# Autodesk Inventor assembly: fork_left
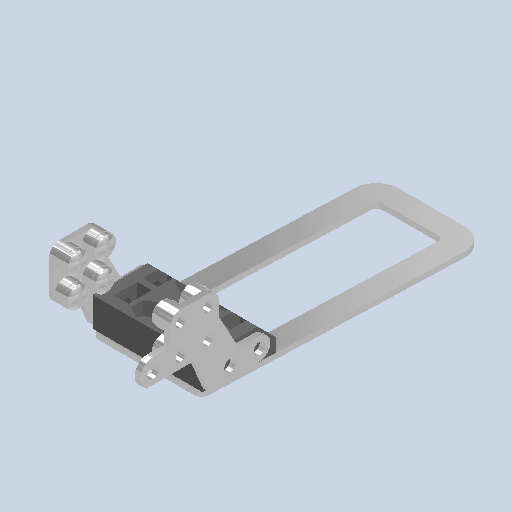
[picture p0: Inventor's stored thumbnail of the model, 512x512]
Saved by Autodesk Inventor 2024.1 (Build 281209000, 209)
## iProperties
Created: 2025-01-18
Part Number: fork_left
Document SubType Name: Assembly
Designer: hibik
Author: hibik
## Documents named in this file (6)
- C:\Users\hibik\Documents\Robomech\RESCUE\ORCA\hard\fork\left\fork_left.iam
- C:\Users\hibik\Documents\Robomech\RESCUE\ORCA\hard\fork\left\fork_middle_left.ipt
- C:\Users\hibik\Documents\Robomech\RESCUE\ORCA\hard\fork\left\fork_inside_left.ipt
- C:\Users\hibik\Documents\Robomech\RESCUE\ORCA\hard\fork\left\fork_outside_left.ipt
- C:\Users\hibik\Documents\Robomech\RESCUE\ORCA\hard\fork\left\bearing_3_6_2.5_left.ipt
- C:\Users\hibik\Documents\Robomech\RESCUE\ORCA\hard\fork\left\fork_fork_left.ipt
## Components (12 placed, 5 different names)
1. fork_middle_left:1 — 挿入:4, 挿入:3, 挿入:2, 挿入:1, 挿入:16, 挿入:15, 挿入:14, 挿入:13
2. fork_inside_left:1 — 挿入:4, 挿入:3, 挿入:9, 挿入:10, 挿入:12, 挿入:11
3. fork_outside_left:1 — 挿入:2, 挿入:1, 挿入:5, 挿入:6, 挿入:8, 挿入:7
4. bearing_3_6_2.5_left:1 — 挿入:5
5. bearing_3_6_2.5_left:2 — 挿入:6
6. bearing_3_6_2.5_left:3 — 挿入:8
7. bearing_3_6_2.5_left:4 — 挿入:7
8. bearing_3_6_2.5_left:5 — 挿入:9
9. bearing_3_6_2.5_left:6 — 挿入:10
10. bearing_3_6_2.5_left:7 — 挿入:12
11. bearing_3_6_2.5_left:8 — 挿入:11
12. fork_fork_left:1 — 挿入:16, 挿入:15, 挿入:14, 挿入:13
## Relationships (16: Insert 16)
- 挿入:4 [Insert]: fork_middle_left:1 ↔ fork_inside_left:1
- 挿入:3 [Insert]: fork_middle_left:1 ↔ fork_inside_left:1
- 挿入:2 [Insert]: fork_middle_left:1 ↔ fork_outside_left:1
- 挿入:1 [Insert]: fork_middle_left:1 ↔ fork_outside_left:1
- 挿入:5 [Insert]: fork_outside_left:1 ↔ bearing_3_6_2.5_left:1
- 挿入:6 [Insert]: fork_outside_left:1 ↔ bearing_3_6_2.5_left:2
- 挿入:8 [Insert]: fork_outside_left:1 ↔ bearing_3_6_2.5_left:3
- 挿入:7 [Insert]: fork_outside_left:1 ↔ bearing_3_6_2.5_left:4
- 挿入:9 [Insert]: fork_inside_left:1 ↔ bearing_3_6_2.5_left:5
- 挿入:10 [Insert]: fork_inside_left:1 ↔ bearing_3_6_2.5_left:6
- 挿入:12 [Insert]: fork_inside_left:1 ↔ bearing_3_6_2.5_left:7
- 挿入:11 [Insert]: fork_inside_left:1 ↔ bearing_3_6_2.5_left:8
- 挿入:16 [Insert]: fork_middle_left:1 ↔ fork_fork_left:1
- 挿入:15 [Insert]: fork_middle_left:1 ↔ fork_fork_left:1
- 挿入:14 [Insert]: fork_middle_left:1 ↔ fork_fork_left:1
- 挿入:13 [Insert]: fork_middle_left:1 ↔ fork_fork_left:1
